# Autodesk Inventor assembly: 組合1
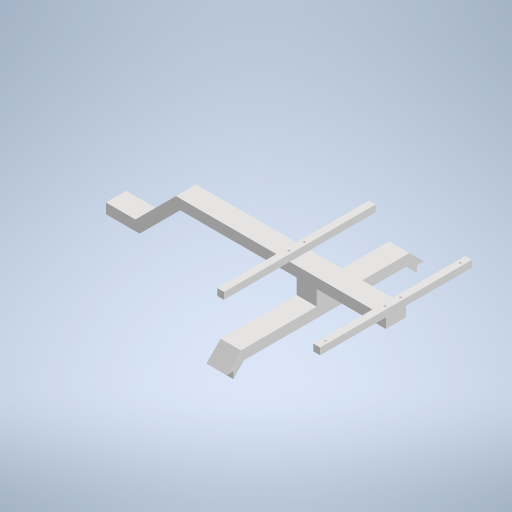
[picture p0: Inventor's stored thumbnail of the model, 512x512]
Saved by Autodesk Inventor 2024 (Build 280153000, 153)
## iProperties
Created: 2024-10-15
Part Number: 組合1
Document SubType Name: Assembly
Designer: jerry
Author: jerry
## Documents named in this file (7)
- C:\Users\jerry\Desktop\Inventor Model\組合1.iam
- C:\Users\jerry\Desktop\Inventor Model\Body Actuator.ipt
- C:\Users\jerry\Desktop\Inventor Model\DOF1.ipt
- C:\Users\jerry\Desktop\Inventor Model\DOF2.ipt
- C:\Users\jerry\Desktop\Inventor Model\DOF3.ipt
- C:\Users\jerry\Desktop\Inventor Model\DOF4.ipt
- C:\Users\jerry\Desktop\Inventor Model\DOF5.ipt
## Components (6 placed, 6 different names)
1. Body Actuator:1 — 齊平:1, 齊平:3
2. DOF1:1 — 齊平:1, 齊平:2
3. DOF2:1 — 齊平:2, 齊平:4
4. DOF3:1 — 齊平:3
5. DOF4:1 — 齊平:4, 齊平:5
6. DOF5:1 — 齊平:5
## Relationships (5: Flush 5)
- 齊平:1 [Flush]: Body Actuator:1 ↔ DOF1:1
- 齊平:2 [Flush]: DOF1:1 ↔ DOF2:1
- 齊平:3 [Flush]: Body Actuator:1 ↔ DOF3:1
- 齊平:4 [Flush]: DOF2:1 ↔ DOF4:1
- 齊平:5 [Flush]: DOF4:1 ↔ DOF5:1
